# Autodesk Inventor assembly: sensor_subassy
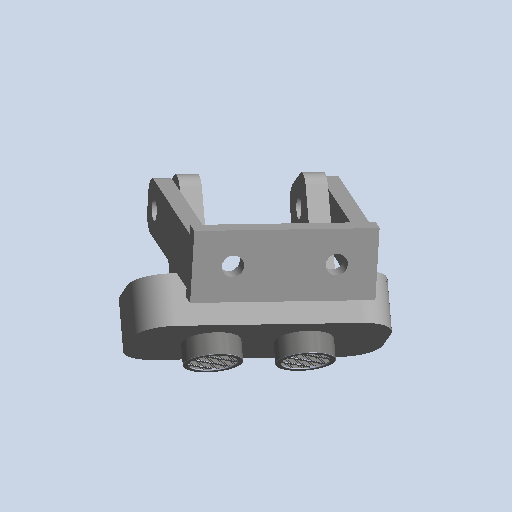
[picture p0: Inventor's stored thumbnail of the model, 512x512]
Saved by Autodesk Inventor 2026 (Build 300175050, 175E)
## iProperties
Part Number: sensor_subassy
Document SubType Name: Assembly
Designer: Kartik
Mass: 36.7326 g
Surface Area: 282.998 cm^2
Volume: 36.7326 cm^3
Density: 1 g/cm^3
Author: Kartik
## Documents named in this file (5)
- D:\Kartik\Projects\AMR\CAD\2 Sub-assembly\sensor_subassy.iam
- D:\Kartik\Projects\AMR\CAD\4 Boughtouts\hc-sr04-ultrasonic-sensor-12\Ultrasonic sensor\Ultrasonic sensor\Ultrasonic sensor.ipt
- D:\Kartik\Projects\AMR\CAD\3 Parts\sensor_cover_ultrasonic.ipt
- D:\Kartik\Projects\AMR\CAD\3 Parts\sensor_cover_ultrasonic_2.ipt
- D:\Kartik\Projects\AMR\CAD\3 Parts\sensor_cover_ultrasonic_3.ipt
## Components (4 placed, 4 different names)
1. Ultrasonic sensor:1 — Mate:1, Mate:2, Mate:3
2. sensor_cover_ultrasonic:1 — Mate:1, Mate:2, Mate:3, Mate:4, Mate:5, Mate:6
3. sensor_cover_ultrasonic_2:1 — Mate:4, Mate:5, Mate:6, Mate:7, Mate:8
4. sensor_cover_ultrasonic_3:1 — Mate:7, Mate:8
## Relationships (8: Mate 8)
- Mate:1: Ultrasonic sensor:1 ↔ sensor_cover_ultrasonic:1
- Mate:2: Ultrasonic sensor:1 ↔ sensor_cover_ultrasonic:1
- Mate:3: Ultrasonic sensor:1 ↔ sensor_cover_ultrasonic:1
- Mate:4: sensor_cover_ultrasonic:1 ↔ sensor_cover_ultrasonic_2:1
- Mate:5: sensor_cover_ultrasonic:1 ↔ sensor_cover_ultrasonic_2:1
- Mate:6: sensor_cover_ultrasonic:1 ↔ sensor_cover_ultrasonic_2:1
- Mate:7: sensor_cover_ultrasonic_2:1 ↔ sensor_cover_ultrasonic_3:1
- Mate:8: sensor_cover_ultrasonic_2:1 ↔ sensor_cover_ultrasonic_3:1
